# Autodesk Inventor assembly: SpecSUPERGEAR
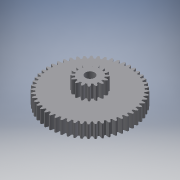
[picture p0: Inventor's stored thumbnail of the model, 180x180]
Saved by Autodesk Inventor 2016 (Build 200138000, 138)
## iProperties
Created: 2018-03-03
Part Number: SpecSUPERGEAR
Document SubType Name: Assembly
Designer: Simon
Author: Simon
## Documents named in this file (3)
- D:\Cad\Gymnasieprojekt\SpecSUPERGEAR.iam
- D:\Cad\Gymnasieprojekt\SUPERGEAR2.ipt
- D:\Cad\Gymnasieprojekt\SUPERGEAR12.ipt
## Components (2 placed, 2 different names)
1. SUPERGEAR2:1 — Insert:1
2. SUPERGEAR12:1 — Insert:1
## Relationships (1: Insert 1)
- Insert:1: SUPERGEAR2:1 ↔ SUPERGEAR12:1
